# Autodesk Inventor assembly: Assembly1
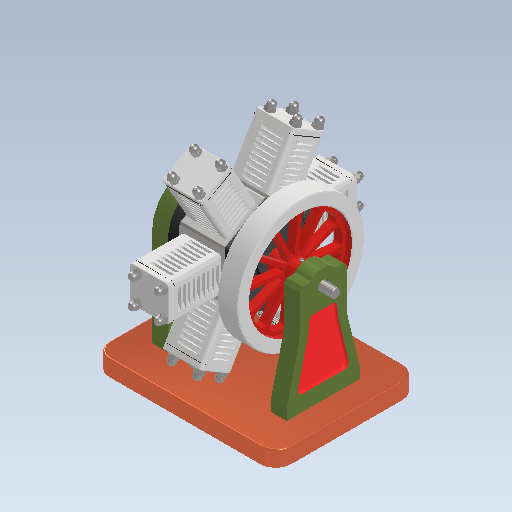
[picture p0: Inventor's stored thumbnail of the model, 512x512]
Saved by Autodesk Inventor 2020 (Build 240168000, 168)
## iProperties
Created: 2020-08-16
Part Number: Assembly1
Document SubType Name: Assembly
Designer: benny
Author: benny
## Documents named in this file (23)
- C:\Users\benny\Desktop\importantmajorprojecthev_june\engine\assembly\BENNY S L_JUNE BATCH_Assembly.iam
- C:\Users\benny\Desktop\importantmajorprojecthev_june\engine\crankshaft assembly\BENNY S L_JUNE BATCH_crankshaft assembly.iam
- C:\Users\benny\Desktop\importantmajorprojecthev_june\engine\others\Benny S L_JUNE BATCH_stand\Benny S L_JUNE BATCH_stand.ipt
- C:\Users\benny\Desktop\importantmajorprojecthev_june\engine\others\Benny S L_JUNE BATCH_bearing holder.ipt
- C:\Users\benny\Desktop\importantmajorprojecthev_june\engine\others\Benny S L_JUNE BATCH_bearing stand.ipt
- C:\Users\benny\Documents\Inventor\Content Center Files\R2020\en-US\ISO 4762(2)\ISO 4762 - M10 x 25ISO.ipt
- C:\Users\benny\Documents\Inventor\Content Center Files\R2020\en-US\Parker HB 125HBL\Parker Hose Barb to Male Pipe 125HBL 125HBL-4-2.ipt
- C:\Users\benny\Desktop\importantmajorprojecthev_june\engine\others\Benny S L_JUNE BATCH_valve housing\Benny S L_JUNE BATCH_valve housing.ipt
- C:\Users\benny\Desktop\importantmajorprojecthev_june\engine\others\Benny S L_JUNE BATCH_valve\Benny S L_JUNE BATCH_valve.ipt
- C:\Users\benny\Desktop\importantmajorprojecthev_june\engine\others\Benny S L_JUNE BATCH_crank case set\Benny S L_JUNE BATCH_crankcase.ipt
- C:\Users\benny\Documents\Inventor\Content Center Files\R2020\en-US\ISO 4762(2)\ISO 4762 - M6 x 45ISO.ipt
- C:\Users\benny\Desktop\importantmajorprojecthev_june\engine\assembly\BENNY S L_JUNE BATCH_Assembly2.iam
- C:\Users\benny\Documents\Inventor\Content Center Files\R2020\en-US\DIN BEARING(1)\DIN 625 SKF - SKF 6001.ipt
- C:\Users\benny\Desktop\importantmajorprojecthev_june\engine\others\Benny S L_JUNE BATCH_connecting rod hub.ipt
- C:\Users\benny\Desktop\importantmajorprojecthev_june\engine\others\Benny S L_JUNE BATCH_flywheel.ipt
- C:\Users\benny\Desktop\importantmajorprojecthev_june\engine\others\Benny S L_JUNE BATCH_connecting rod.ipt
- C:\Users\benny\Desktop\importantmajorprojecthev_june\engine\piston assembly\Benny S L_JUNE BATCH_Assembly piston.iam
- C:\Users\benny\Documents\Inventor\Content Center Files\R2020\en-US\ISO 2338(2)\ISO 2338 - 5 h8 x 16.ipt
- C:\Users\benny\Desktop\importantmajorprojecthev_june\engine\others\Benny S L_JUNE BATCH_crank case set\Benny S L_JUNE BATCH_crank case cover.ipt
- C:\Users\benny\Desktop\importantmajorprojecthev_june\engine\others\Benny S L_JUNE BATCH_crank case set\Benny S L_JUNE BATCH_crankcase gasket.ipt
- C:\Users\benny\Documents\Inventor\Content Center Files\R2020\en-US\ISO 7045  H\ISO 7045 - M6 x 16 - 4.8 - H - ISO.ipt
- C:\Users\benny\Documents\Inventor\Content Center Files\R2020\en-US\DIN 472(2)\DIN 472 - 28x1.2.ipt
- C:\Users\benny\Documents\Inventor\Content Center Files\R2020\en-US\ISO 4028\ISO 4028 - M5 x 8 - ISO.ipt
## Components (57 placed, 22 different names)
1. BENNY S L_JUNE BATCH_crankshaft assembly:1 [sub-assembly] — Mate:93, Mate:94, Mate:95, Mate:96, Mate:97, Mate:98, Mate:117, Mate:118, Mate:119, Mate:121, Mate:128
2. Benny S L_JUNE BATCH_stand:1 — Mate:1, Mate:2, Mate:3, Mate:4, Mate:5, Mate:6, Mate:7, Mate:8, Mate:9, Mate:10, Mate:11, Mate:12, Mate:13, Mate:14
3. Benny S L_JUNE BATCH_bearing holder:1 — Mate:4, Mate:5, Mate:6, Mate:120, Mate:122, Mate:126
4. Benny S L_JUNE BATCH_bearing stand:1 — Mate:1, Mate:2, Mate:3, Mate:15, Mate:16, Mate:17, Mate:18, Mate:25, Mate:26, Mate:27, Mate:28, Mate:29, Mate:30, Mate:31, Mate:32, Mate:33, Mate:34, Mate:35, Mate:36
5. ISO 4762 M10 x 25:1 — Mate:11, Mate:12
6. ISO 4762 M10 x 25:2 — Mate:13, Mate:14
7. ISO 4762 M10 x 25:3 — Mate:9, Mate:10
8. ISO 4762 M10 x 25:4 — Mate:7, Mate:8
9. Parker Hose Barb to Male Pipe 125HBL 125HBL-4-2:1 — Mate:15, Mate:19
10. Benny S L_JUNE BATCH_valve housing:1 — Mate:16, Mate:17, Mate:18, Mate:19, Mate:20, Mate:21, Mate:23, Mate:24
11. Benny S L_JUNE BATCH_valve:1 — Mate:20, Mate:21, Mate:22, Mate:93
12. Benny S L_JUNE BATCH_crankcase:1 — Mate:22, Mate:23, Mate:24, Mate:37, Mate:38, Mate:39, Mate:73, Mate:76, Mate:77, Mate:99, Mate:100
13. ISO 4762 M6 x 45:1 — Mate:35, Mate:36
14. ISO 4762 M6 x 45:2 — Mate:33, Mate:34
15. ISO 4762 M6 x 45:3 — Mate:31, Mate:32
16. ISO 4762 M6 x 45:4 — Mate:29, Mate:30
17. ISO 4762 M6 x 45:5 — Mate:27, Mate:28
18. ISO 4762 M6 x 45:6 — Mate:25, Mate:26
19. DIN 625 SKF SKF 6001:1 — Mate:76, Mate:77, Mate:95
20. DIN 625 SKF SKF 6001:2 — Mate:96, Mate:97
21. DIN 625 SKF SKF 6001:3 — Mate:118, Mate:119, Mate:120
22. Benny S L_JUNE BATCH_connecting rod hub:1 — Mate:52, Mate:53, Mate:54, Mate:55, Mate:56, Mate:57, Mate:58, Mate:59, Mate:60, Mate:61, Mate:62, Mate:63, Mate:64, Mate:65, Mate:66, Mate:68, Mate:69, Flush:1, Flush:2, Flush:3, Flush:4, Flush:5, Flush:6, Mate:94
23. Benny S L_JUNE BATCH_flywheel:1 — Mate:117, Mate:126, Mate:127
24. Benny S L_JUNE BATCH_connecting rod:1 — Mate:56, Mate:57, Mate:83, Mate:84, Mate:85
25. Benny S L_JUNE BATCH_connecting rod:2 — Mate:62, Mate:63, Mate:79, Mate:86
26. Benny S L_JUNE BATCH_connecting rod:3 — Mate:60, Mate:61, Mate:78, Mate:87
27. Benny S L_JUNE BATCH_connecting rod:4 — Mate:58, Mate:59, Mate:67, Mate:82, Mate:88
28. Benny S L_JUNE BATCH_connecting rod:5 — Mate:52, Mate:53, Mate:89, Mate:90
29. Benny S L_JUNE BATCH_connecting rod:6 — Mate:54, Mate:55, Mate:91, Mate:92
30. Benny S L_JUNE BATCH_Assembly piston:1 [sub-assembly] — Mate:82, Mate:88, Mate:124
31. Benny S L_JUNE BATCH_Assembly piston:2 [sub-assembly] — Mate:71, Mate:78, Mate:87
32. Benny S L_JUNE BATCH_Assembly piston:3 [sub-assembly] — Mate:73, Mate:83, Mate:84, Mate:85
33. Benny S L_JUNE BATCH_Assembly piston:4 [sub-assembly] — Mate:89, Mate:90, Mate:125
34. Benny S L_JUNE BATCH_Assembly piston:5 [sub-assembly] — Mate:79, Mate:86, Mate:123
35. ISO 2338 5 h8 x 16:1 — Mate:68, Flush:3
36. ISO 2338 5 h8 x 16:2 — Mate:66, Flush:5
37. ISO 2338 5 h8 x 16:3 — Mate:67, Flush:4
38. ISO 2338 5 h8 x 16:4 — Mate:65, Flush:2
39. ISO 2338 5 h8 x 16:5 — Mate:64, Flush:1
40. ISO 2338 5 h8 x 16:6 — Mate:69, Flush:6
41. Benny S L_JUNE BATCH_Assembly piston:6 [sub-assembly] — Mate:75, Mate:91, Mate:92
42. Benny S L_JUNE BATCH_crank case cover:1 — Mate:98, Mate:99, Mate:100, Mate:101, Mate:102, Mate:103, Mate:104, Mate:106, Mate:107, Mate:108, Mate:109, Mate:110, Mate:111, Mate:112
43. Benny S L_JUNE BATCH_crankcase gasket:1 — Mate:101, Mate:102, Mate:103, Mate:105, Mate:113, Mate:114, Mate:115, Mate:116
44. ISO 7045 H M6 x 16 - 4.8 - H:1 — Mate:109, Mate:112
45. ISO 7045 H M6 x 16 - 4.8 - H:2 — Mate:106, Mate:111
46. ISO 7045 H M6 x 16 - 4.8 - H:3 — Mate:110, Mate:115
47. ISO 7045 H M6 x 16 - 4.8 - H:4 — Mate:104, Mate:105, Mate:113
48. ISO 7045 H M6 x 16 - 4.8 - H:5 — Mate:107, Mate:114
49. ISO 7045 H M6 x 16 - 4.8 - H:6 — Mate:108, Mate:116
50. DIN 472 28x1.2:1 — Mate:121, Mate:122
51. ISO 4028 M5 x 8:1 — Mate:127, Mate:128
52. BENNY S L_JUNE BATCH_Assembly2:1 [sub-assembly] — Mate:37, Mate:38, Mate:39, Mate:71
53. BENNY S L_JUNE BATCH_Assembly2:7 [sub-assembly] — Mate:124
54. BENNY S L_JUNE BATCH_Assembly2:8 [sub-assembly]
55. BENNY S L_JUNE BATCH_Assembly2:9 [sub-assembly] — Mate:75
56. BENNY S L_JUNE BATCH_Assembly2:10 [sub-assembly] — Mate:125
57. BENNY S L_JUNE BATCH_Assembly2:11 [sub-assembly] — Mate:123
## Component patterns: (6 elements, first: BENNY S L_JUNE BATCH_Assembly2:1)
## Relationships (117: Mate 111, Flush 6)
- Mate:1: Benny S L_JUNE BATCH_stand:1 ↔ Benny S L_JUNE BATCH_bearing stand:1
- Mate:2: Benny S L_JUNE BATCH_stand:1 ↔ Benny S L_JUNE BATCH_bearing stand:1
- Mate:3: Benny S L_JUNE BATCH_stand:1 ↔ Benny S L_JUNE BATCH_bearing stand:1
- Mate:4: Benny S L_JUNE BATCH_stand:1 ↔ Benny S L_JUNE BATCH_bearing holder:1
- Mate:5: Benny S L_JUNE BATCH_stand:1 ↔ Benny S L_JUNE BATCH_bearing holder:1
- Mate:6: Benny S L_JUNE BATCH_stand:1 ↔ Benny S L_JUNE BATCH_bearing holder:1
- Mate:7: Benny S L_JUNE BATCH_stand:1 ↔ ISO 4762 M10 x 25:4
- Mate:8: Benny S L_JUNE BATCH_stand:1 ↔ ISO 4762 M10 x 25:4
- Mate:9: Benny S L_JUNE BATCH_stand:1 ↔ ISO 4762 M10 x 25:3
- Mate:10: Benny S L_JUNE BATCH_stand:1 ↔ ISO 4762 M10 x 25:3
- Mate:11: Benny S L_JUNE BATCH_stand:1 ↔ ISO 4762 M10 x 25:1
- Mate:12: Benny S L_JUNE BATCH_stand:1 ↔ ISO 4762 M10 x 25:1
- Mate:13: Benny S L_JUNE BATCH_stand:1 ↔ ISO 4762 M10 x 25:2
- Mate:14: Benny S L_JUNE BATCH_stand:1 ↔ ISO 4762 M10 x 25:2
- Mate:15: Benny S L_JUNE BATCH_bearing stand:1 ↔ Parker Hose Barb to Male Pipe 125HBL 125HBL-4-2:1
- Mate:16: Benny S L_JUNE BATCH_bearing stand:1 ↔ Benny S L_JUNE BATCH_valve housing:1
- Mate:17: Benny S L_JUNE BATCH_bearing stand:1 ↔ Benny S L_JUNE BATCH_valve housing:1
- Mate:18: Benny S L_JUNE BATCH_bearing stand:1 ↔ Benny S L_JUNE BATCH_valve housing:1
- Mate:19: Parker Hose Barb to Male Pipe 125HBL 125HBL-4-2:1 ↔ Benny S L_JUNE BATCH_valve housing:1
- Mate:20: Benny S L_JUNE BATCH_valve housing:1 ↔ Benny S L_JUNE BATCH_valve:1
- Mate:21: Benny S L_JUNE BATCH_valve housing:1 ↔ Benny S L_JUNE BATCH_valve:1
- Mate:22: Benny S L_JUNE BATCH_valve:1 ↔ Benny S L_JUNE BATCH_crankcase:1
- Mate:23: Benny S L_JUNE BATCH_valve housing:1 ↔ Benny S L_JUNE BATCH_crankcase:1
- Mate:24: Benny S L_JUNE BATCH_valve housing:1 ↔ Benny S L_JUNE BATCH_crankcase:1
- Mate:25: Benny S L_JUNE BATCH_bearing stand:1 ↔ ISO 4762 M6 x 45:6
- Mate:26: Benny S L_JUNE BATCH_bearing stand:1 ↔ ISO 4762 M6 x 45:6
- Mate:27: Benny S L_JUNE BATCH_bearing stand:1 ↔ ISO 4762 M6 x 45:5
- Mate:28: Benny S L_JUNE BATCH_bearing stand:1 ↔ ISO 4762 M6 x 45:5
- Mate:29: Benny S L_JUNE BATCH_bearing stand:1 ↔ ISO 4762 M6 x 45:4
- Mate:30: Benny S L_JUNE BATCH_bearing stand:1 ↔ ISO 4762 M6 x 45:4
- Mate:31: Benny S L_JUNE BATCH_bearing stand:1 ↔ ISO 4762 M6 x 45:3
- Mate:32: Benny S L_JUNE BATCH_bearing stand:1 ↔ ISO 4762 M6 x 45:3
- Mate:33: Benny S L_JUNE BATCH_bearing stand:1 ↔ ISO 4762 M6 x 45:2
- Mate:34: Benny S L_JUNE BATCH_bearing stand:1 ↔ ISO 4762 M6 x 45:2
- Mate:35: Benny S L_JUNE BATCH_bearing stand:1 ↔ ISO 4762 M6 x 45:1
- Mate:36: Benny S L_JUNE BATCH_bearing stand:1 ↔ ISO 4762 M6 x 45:1
- Mate:37: Benny S L_JUNE BATCH_crankcase:1 ↔ BENNY S L_JUNE BATCH_Assembly2:1
- Mate:38: Benny S L_JUNE BATCH_crankcase:1 ↔ BENNY S L_JUNE BATCH_Assembly2:1
- Mate:39: Benny S L_JUNE BATCH_crankcase:1 ↔ BENNY S L_JUNE BATCH_Assembly2:1
- Mate:52: Benny S L_JUNE BATCH_connecting rod hub:1 ↔ Benny S L_JUNE BATCH_connecting rod:5
- Mate:53: Benny S L_JUNE BATCH_connecting rod hub:1 ↔ Benny S L_JUNE BATCH_connecting rod:5
- Mate:54: Benny S L_JUNE BATCH_connecting rod hub:1 ↔ Benny S L_JUNE BATCH_connecting rod:6
- Mate:55: Benny S L_JUNE BATCH_connecting rod hub:1 ↔ Benny S L_JUNE BATCH_connecting rod:6
- Mate:56: Benny S L_JUNE BATCH_connecting rod hub:1 ↔ Benny S L_JUNE BATCH_connecting rod:1
- Mate:57: Benny S L_JUNE BATCH_connecting rod hub:1 ↔ Benny S L_JUNE BATCH_connecting rod:1
- Mate:58: Benny S L_JUNE BATCH_connecting rod hub:1 ↔ Benny S L_JUNE BATCH_connecting rod:4
- Mate:59: Benny S L_JUNE BATCH_connecting rod hub:1 ↔ Benny S L_JUNE BATCH_connecting rod:4
- Mate:60: Benny S L_JUNE BATCH_connecting rod hub:1 ↔ Benny S L_JUNE BATCH_connecting rod:3
- Mate:61: Benny S L_JUNE BATCH_connecting rod hub:1 ↔ Benny S L_JUNE BATCH_connecting rod:3
- Mate:62: Benny S L_JUNE BATCH_connecting rod hub:1 ↔ Benny S L_JUNE BATCH_connecting rod:2
- Mate:63: Benny S L_JUNE BATCH_connecting rod hub:1 ↔ Benny S L_JUNE BATCH_connecting rod:2
- Mate:64: Benny S L_JUNE BATCH_connecting rod hub:1 ↔ ISO 2338 5 h8 x 16:5
- Mate:65: Benny S L_JUNE BATCH_connecting rod hub:1 ↔ ISO 2338 5 h8 x 16:4
- Mate:66: Benny S L_JUNE BATCH_connecting rod hub:1 ↔ ISO 2338 5 h8 x 16:2
- Mate:67: Benny S L_JUNE BATCH_connecting rod:4 ↔ ISO 2338 5 h8 x 16:3
- Mate:68: Benny S L_JUNE BATCH_connecting rod hub:1 ↔ ISO 2338 5 h8 x 16:1
- Mate:69: Benny S L_JUNE BATCH_connecting rod hub:1 ↔ ISO 2338 5 h8 x 16:6
- Flush:1: Benny S L_JUNE BATCH_connecting rod hub:1 ↔ ISO 2338 5 h8 x 16:5
- Flush:2: Benny S L_JUNE BATCH_connecting rod hub:1 ↔ ISO 2338 5 h8 x 16:4
- Flush:3: Benny S L_JUNE BATCH_connecting rod hub:1 ↔ ISO 2338 5 h8 x 16:1
- Flush:4: Benny S L_JUNE BATCH_connecting rod hub:1 ↔ ISO 2338 5 h8 x 16:3
- Flush:5: Benny S L_JUNE BATCH_connecting rod hub:1 ↔ ISO 2338 5 h8 x 16:2
- Flush:6: Benny S L_JUNE BATCH_connecting rod hub:1 ↔ ISO 2338 5 h8 x 16:6
- Mate:71: Benny S L_JUNE BATCH_Assembly piston:2 ↔ BENNY S L_JUNE BATCH_Assembly2:1
- Mate:73: Benny S L_JUNE BATCH_crankcase:1 ↔ Benny S L_JUNE BATCH_Assembly piston:3
- Mate:75: Benny S L_JUNE BATCH_Assembly piston:6 ↔ BENNY S L_JUNE BATCH_Assembly2:9
- Mate:76: Benny S L_JUNE BATCH_crankcase:1 ↔ DIN 625 SKF SKF 6001:1
- Mate:77: Benny S L_JUNE BATCH_crankcase:1 ↔ DIN 625 SKF SKF 6001:1
- Mate:78 (-5 mm): Benny S L_JUNE BATCH_connecting rod:3 ↔ Benny S L_JUNE BATCH_Assembly piston:2
- Mate:79 (-5 mm): Benny S L_JUNE BATCH_connecting rod:2 ↔ Benny S L_JUNE BATCH_Assembly piston:5
- Mate:82 (-5 mm): Benny S L_JUNE BATCH_connecting rod:4 ↔ Benny S L_JUNE BATCH_Assembly piston:1
- Mate:83 (-5 mm): Benny S L_JUNE BATCH_connecting rod:1 ↔ Benny S L_JUNE BATCH_Assembly piston:3
- Mate:84 (-5 mm): Benny S L_JUNE BATCH_connecting rod:1 ↔ Benny S L_JUNE BATCH_Assembly piston:3
- Mate:85: Benny S L_JUNE BATCH_connecting rod:1 ↔ Benny S L_JUNE BATCH_Assembly piston:3
- Mate:86: Benny S L_JUNE BATCH_connecting rod:2 ↔ Benny S L_JUNE BATCH_Assembly piston:5
- Mate:87: Benny S L_JUNE BATCH_connecting rod:3 ↔ Benny S L_JUNE BATCH_Assembly piston:2
- Mate:88: Benny S L_JUNE BATCH_connecting rod:4 ↔ Benny S L_JUNE BATCH_Assembly piston:1
- Mate:89 (-5 mm): Benny S L_JUNE BATCH_connecting rod:5 ↔ Benny S L_JUNE BATCH_Assembly piston:4
- Mate:90: Benny S L_JUNE BATCH_connecting rod:5 ↔ Benny S L_JUNE BATCH_Assembly piston:4
- Mate:91 (-5 mm): Benny S L_JUNE BATCH_connecting rod:6 ↔ Benny S L_JUNE BATCH_Assembly piston:6
- Mate:92: Benny S L_JUNE BATCH_connecting rod:6 ↔ Benny S L_JUNE BATCH_Assembly piston:6
- Mate:93: BENNY S L_JUNE BATCH_crankshaft assembly:1 ↔ Benny S L_JUNE BATCH_valve:1
- Mate:94: BENNY S L_JUNE BATCH_crankshaft assembly:1 ↔ Benny S L_JUNE BATCH_connecting rod hub:1
- Mate:95: BENNY S L_JUNE BATCH_crankshaft assembly:1 ↔ DIN 625 SKF SKF 6001:1
- Mate:96: BENNY S L_JUNE BATCH_crankshaft assembly:1 ↔ DIN 625 SKF SKF 6001:2
- Mate:97: BENNY S L_JUNE BATCH_crankshaft assembly:1 ↔ DIN 625 SKF SKF 6001:2
- Mate:98: BENNY S L_JUNE BATCH_crankshaft assembly:1 ↔ Benny S L_JUNE BATCH_crank case cover:1
- Mate:99: Benny S L_JUNE BATCH_crankcase:1 ↔ Benny S L_JUNE BATCH_crank case cover:1
- Mate:100: Benny S L_JUNE BATCH_crankcase:1 ↔ Benny S L_JUNE BATCH_crank case cover:1
- Mate:101: Benny S L_JUNE BATCH_crank case cover:1 ↔ Benny S L_JUNE BATCH_crankcase gasket:1
- Mate:102: Benny S L_JUNE BATCH_crank case cover:1 ↔ Benny S L_JUNE BATCH_crankcase gasket:1
- Mate:103: Benny S L_JUNE BATCH_crank case cover:1 ↔ Benny S L_JUNE BATCH_crankcase gasket:1
- Mate:104: Benny S L_JUNE BATCH_crank case cover:1 ↔ ISO 7045 H M6 x 16 - 4.8 - H:4
- Mate:105: Benny S L_JUNE BATCH_crankcase gasket:1 ↔ ISO 7045 H M6 x 16 - 4.8 - H:4
- Mate:106: Benny S L_JUNE BATCH_crank case cover:1 ↔ ISO 7045 H M6 x 16 - 4.8 - H:2
- Mate:107: Benny S L_JUNE BATCH_crank case cover:1 ↔ ISO 7045 H M6 x 16 - 4.8 - H:5
- Mate:108: Benny S L_JUNE BATCH_crank case cover:1 ↔ ISO 7045 H M6 x 16 - 4.8 - H:6
- Mate:109: Benny S L_JUNE BATCH_crank case cover:1 ↔ ISO 7045 H M6 x 16 - 4.8 - H:1
- Mate:110: Benny S L_JUNE BATCH_crank case cover:1 ↔ ISO 7045 H M6 x 16 - 4.8 - H:3
- Mate:111: Benny S L_JUNE BATCH_crank case cover:1 ↔ ISO 7045 H M6 x 16 - 4.8 - H:2
- Mate:112: Benny S L_JUNE BATCH_crank case cover:1 ↔ ISO 7045 H M6 x 16 - 4.8 - H:1
- Mate:113: Benny S L_JUNE BATCH_crankcase gasket:1 ↔ ISO 7045 H M6 x 16 - 4.8 - H:4
- Mate:114: Benny S L_JUNE BATCH_crankcase gasket:1 ↔ ISO 7045 H M6 x 16 - 4.8 - H:5
- Mate:115: Benny S L_JUNE BATCH_crankcase gasket:1 ↔ ISO 7045 H M6 x 16 - 4.8 - H:3
- Mate:116: Benny S L_JUNE BATCH_crankcase gasket:1 ↔ ISO 7045 H M6 x 16 - 4.8 - H:6
- Mate:117: BENNY S L_JUNE BATCH_crankshaft assembly:1 ↔ Benny S L_JUNE BATCH_flywheel:1
- Mate:118: BENNY S L_JUNE BATCH_crankshaft assembly:1 ↔ DIN 625 SKF SKF 6001:3
- Mate:119: BENNY S L_JUNE BATCH_crankshaft assembly:1 ↔ DIN 625 SKF SKF 6001:3
- Mate:120: Benny S L_JUNE BATCH_bearing holder:1 ↔ DIN 625 SKF SKF 6001:3
- Mate:121: BENNY S L_JUNE BATCH_crankshaft assembly:1 ↔ DIN 472 28x1.2:1
- Mate:122: Benny S L_JUNE BATCH_bearing holder:1 ↔ DIN 472 28x1.2:1
- Mate:123: Benny S L_JUNE BATCH_Assembly piston:5 ↔ BENNY S L_JUNE BATCH_Assembly2:11
- Mate:124: Benny S L_JUNE BATCH_Assembly piston:1 ↔ BENNY S L_JUNE BATCH_Assembly2:7
- Mate:125: Benny S L_JUNE BATCH_Assembly piston:4 ↔ BENNY S L_JUNE BATCH_Assembly2:10
- Mate:126 (2.5 mm): Benny S L_JUNE BATCH_bearing holder:1 ↔ Benny S L_JUNE BATCH_flywheel:1
- Mate:127: Benny S L_JUNE BATCH_flywheel:1 ↔ ISO 4028 M5 x 8:1
- Mate:128 (6 mm): BENNY S L_JUNE BATCH_crankshaft assembly:1 ↔ ISO 4028 M5 x 8:1
